# Autodesk Inventor assembly: vida_mili_montaj
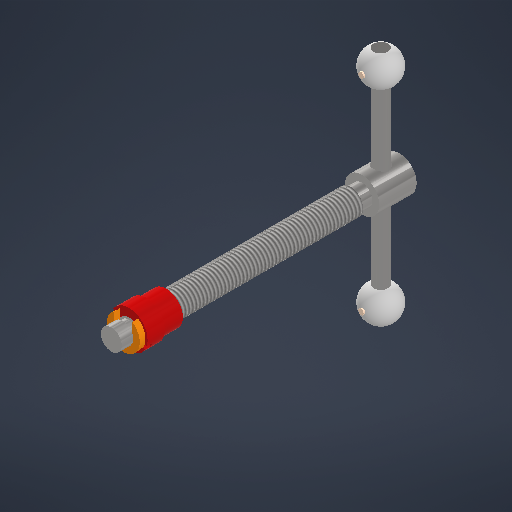
[picture p0: Inventor's stored thumbnail of the model, 512x512]
Saved by Autodesk Inventor 2025.4 (Build 294407000, 407)
## iProperties
Created: 2026-06-20
Part Number: vida_mili_montaj
Document SubType Name: Weldment
Designer: yigithan
Weld Material: Welded Aluminum-6061
Author: yigithan
## Documents named in this file (7)
- C:\Users\yigithan\Desktop\mengene\vida_mili_montaj.iam
- C:\Users\yigithan\Desktop\mengene\parca4.ipt
- C:\Users\yigithan\Desktop\mengene\parca7.ipt
- C:\Users\yigithan\Desktop\mengene\parca8.ipt
- C:\Users\yigithan\Desktop\mengene\parça3.ipt
- C:\Users\yigithan\Desktop\mengene\parça5.ipt
- C:\Users\yigithan\Desktop\mengene\parça6.ipt
## Components (8 placed, 6 different names)
1. parca4:1 — Mate:1, Mate:2, Mate:3, Mate:4, Mate:5, Mate:6
2. parca7:1 — Mate:3, Mate:4, Insert:2
3. parca8:1 — Insert:2
4. parça3:1 — Mate:1, Insert:3, Insert:4
5. parça5:1 — Insert:3
6. parça6:1 — Insert:4
7. parca7:2 — Mate:5, Mate:6, Insert:1
8. parca8:2 — Insert:1
## Relationships (10: Mate 6, Insert 4)
- Mate:1: parca4:1 ↔ parça3:1
- Mate:2 (-65.09 mm): parca4:1
- Mate:3: parca4:1 ↔ parca7:1
- Mate:4: parca4:1 ↔ parca7:1
- Mate:5: parca4:1 ↔ parca7:2
- Mate:6: parca4:1 ↔ parca7:2
- Insert:1: parca7:2 ↔ parca8:2
- Insert:2: parca7:1 ↔ parca8:1
- Insert:3: parça3:1 ↔ parça5:1
- Insert:4: parça3:1 ↔ parça6:1
